# Autodesk Inventor assembly: 217-2 Stage Versaplanetary STEP
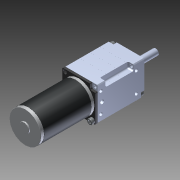
[picture p0: Inventor's stored thumbnail of the model, 180x180]
Saved by Autodesk Inventor 2014 SP1 (Build 180222100, 222)
## iProperties
Created: 2014-01-06
Part Number: 217-2 Stage Versaplanetary STEP
Document SubType Name: Assembly
Designer: Arpan
Title: 217-2 Stage Versaplanetary STEP.STEP
Description: STEP AP214
Creation Date: 2013-12-10
Sending System: SolidWorks 2013
Preprocessor: SwSTEP 2.0
Author: Arpan
## Documents named in this file (18)
- C:\Users\Arpan\Documents\GitHub\2014buildCAD\Shooter\217-2 Stage Versaplanetary STEP.iam
- C:\Users\Arpan\Documents\GitHub\2014buildCAD\Imported Components\217-2 Stage Versaplanetary STEP\217-2625-001 Rev1.ipt
- C:\Users\Arpan\Documents\GitHub\2014buildCAD\Imported Components\217-2 Stage Versaplanetary STEP\217-2625-002 Rev1.ipt
- C:\Users\Arpan\Documents\GitHub\2014buildCAD\Imported Components\217-2 Stage Versaplanetary STEP\217-2625-009 Rev1.ipt
- C:\Users\Arpan\Documents\GitHub\2014buildCAD\Imported Components\217-2 Stage Versaplanetary STEP\217-2816-001 Rev1.ipt
- C:\Users\Arpan\Documents\GitHub\2014buildCAD\Imported Components\217-2 Stage Versaplanetary STEP\217-2625-007 Rev1_Sun_Driver01.ipt
- C:\Users\Arpan\Documents\GitHub\2014buildCAD\Imported Components\217-2 Stage Versaplanetary STEP\217-2625-100.iam
- C:\Users\Arpan\Documents\GitHub\2014buildCAD\Imported Components\217-2 Stage Versaplanetary STEP\217-2822-003 Rev4.ipt
- C:\Users\Arpan\Documents\GitHub\2014buildCAD\Imported Components\217-2 Stage Versaplanetary STEP\217-2625-011 Rev1.ipt
- C:\Users\Arpan\Documents\GitHub\2014buildCAD\Imported Components\217-2 Stage Versaplanetary STEP\SSA_SSA0832-0500ZC.ipt
- C:\Users\Arpan\Documents\GitHub\2014buildCAD\Imported Components\217-2 Stage Versaplanetary STEP\217-2742.ipt
- C:\Users\Arpan\Documents\GitHub\2014buildCAD\Imported Components\217-2 Stage Versaplanetary STEP\SSA_SSA0832-1750ZC.ipt
- C:\Users\Arpan\Documents\GitHub\2014buildCAD\Imported Components\217-2 Stage Versaplanetary STEP\217-2625-018 Rev1_98541A410.ipt
- C:\Users\Arpan\Documents\GitHub\2014buildCAD\Imported Components\217-2 Stage Versaplanetary STEP\217-2625-017 Rev1_9714K61.ipt
- C:\Users\Arpan\Documents\GitHub\2014buildCAD\Imported Components\217-2 Stage Versaplanetary STEP\PINL-M020-006-S.ipt
- C:\Users\Arpan\Documents\GitHub\2014buildCAD\Imported Components\217-2 Stage Versaplanetary STEP\217-3351.ipt
- C:\Users\Arpan\Documents\GitHub\2014buildCAD\Imported Components\217-2 Stage Versaplanetary STEP\217-3106-000 Rev2_NO SUN.iam
- C:\Users\Arpan\Documents\GitHub\2014buildCAD\Shooter\versaplanetarycimoutput.ipt
## Components (21 placed, 21 different names)
1. 217-2625-001 Rev1_1
2. 217-2625-002 Rev1_2 — Mate:1
3. 217-2625-009 Rev1_4
4. 217-2816-001 Rev1_5
5. 217-2625-007 Rev1_Sun_Driver01_6
6. 217-2625-100_7 [sub-assembly]
7. 217-2822-003 Rev4_8
8. 217-2625-011 Rev1_9
9. SSA_SSA0832-0500ZC_10
10. 217-2742_11
11. 217-2742_12 — Mate:2
12. SSA_SSA0832-1750ZC_13
13. SSA_SSA0832-1750ZC_14
14. 217-2625-018 Rev1_98541A410_15
15. 217-2625-017 Rev1_9714K61_16
16. PINL-M020-006-S_17
17. PINL-M020-006-S_18
18. 217-3351_19
19. 217-2816-001 Rev1_20
20. 217-3106-000 Rev2_NO SUN_21 [sub-assembly]
21. versaplanetarycimoutput:1 — Mate:1, Mate:2
## Relationships (2: Mate 2)
- Mate:1: 217-2625-002 Rev1_2 ↔ versaplanetarycimoutput:1
- Mate:2: 217-2742_12 ↔ versaplanetarycimoutput:1
